# Autodesk Inventor assembly: Head plate cap assembly
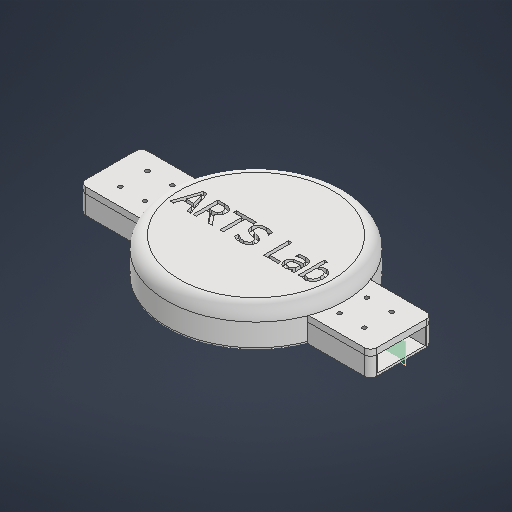
[picture p0: Inventor's stored thumbnail of the model, 512x512]
Saved by Autodesk Inventor 2026.1 (Build 301233000, 233)
## iProperties
Created: 2025-10-24
Part Number: Head plate cap assembly
Document SubType Name: Assembly
Designer: mateo
Author: mateo
## Documents named in this file (4)
- C:\GitHub\In-situ-monitoring-of-powder-bed-fusion-additive-manufacturing\accessories\Head plate cover\Head plate cap assembly.iam
- C:\GitHub\In-situ-monitoring-of-powder-bed-fusion-additive-manufacturing\accessories\Head plate cover\Head Plate Insert.ipt
- C:\GitHub\In-situ-monitoring-of-powder-bed-fusion-additive-manufacturing\accessories\Head plate cover\Metal Head Plate.ipt
- C:\GitHub\In-situ-monitoring-of-powder-bed-fusion-additive-manufacturing\accessories\Head plate cover\Head Plate Cover Cap.ipt
## Components (4 placed, 3 different names)
1. Head Plate Insert:1 — Insert:1
2. Metal Head Plate:1 — Mate:1, Insert:1, Insert:2, Angle:1
3. Head Plate Cover Cap:1 — Mate:1, Mate:2
4. Head Plate Insert:2 — Insert:2
## Relationships (6: Mate 3, Insert 2, Angle 1)
- Mate:1: Metal Head Plate:1 ↔ Head Plate Cover Cap:1
- Insert:1: Head Plate Insert:1 ↔ Metal Head Plate:1
- Insert:2: Metal Head Plate:1 ↔ Head Plate Insert:2
- Mate:2: Head Plate Cover Cap:1
- Mate:3
- Angle:1 (0 deg): Metal Head Plate:1
